# Autodesk Inventor assembly: outside-c-channel
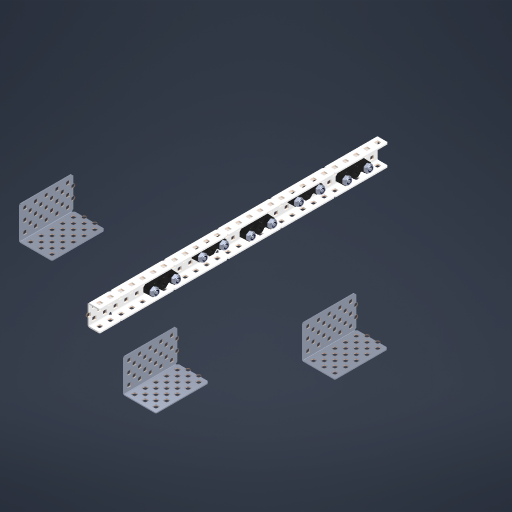
[picture p0: Inventor's stored thumbnail of the model, 512x512]
Saved by Autodesk Inventor 2023 (Build 270158000, 158)
## iProperties
Created: 2023-08-05
Part Number: outside-c-channel
Document SubType Name: Assembly
Designer: srbel
Author: srbel
## Documents named in this file (7)
- C:\CAD\OverUnderCAD\Drive\outside-c-channel.iam
- C:\CAD\OverUnderCAD\VEX-CAD-Inventor-1.4.0\Structure\C Channel\Aluminum 1x2x1\Alu C 1x2x1x27.ipt
- C:\CAD\OverUnderCAD\VEX-CAD-Inventor-1.4.0\Motion\Shaft LS\Bearing Flat.ipt
- C:\CAD\OverUnderCAD\VEX-CAD-Inventor-1.4.0\Structure\Hardware\Screw Steel - Star\SScrew Star Threaded .500.ipt
- C:\CAD\OverUnderCAD\VEX-CAD-Inventor-1.4.0\Structure\Hardware\Nut Thin Nylock.ipt
- C:\CAD\OverUnderCAD\VEX-CAD-Inventor-1.4.0\Structure\Hardware\Screw Steel - Star.ipt
- C:\CAD\OverUnderCAD\VEX-CAD-Inventor-1.4.0\Structure\Angle\Steel\3x3\Steel Angle 3x3x5.ipt
## Components (29 placed, 5 different names)
1. Alu C 1x2x1x27:2 — Insert:1, Insert:2, Insert:3, Insert:4, Insert:5, Insert:6, Insert:7, Insert:8, Insert:21, Insert:22, Insert:23, Insert:24, Insert:25, Insert:26, Insert:27, Insert:28, Insert:29, Insert:30, Insert:31, Insert:32
2. Bearing Flat:1 — Insert:1, Insert:2, Insert:41, Insert:42
3. Bearing Flat:2 — Insert:3, Insert:4, Insert:39, Insert:40
4. Bearing Flat:3 — Insert:5, Insert:6, Insert:37, Insert:38
5. Bearing Flat:4 — Insert:7, Insert:8, Insert:35, Insert:36
6. Bearing Flat:5 — Insert:21, Insert:22, Insert:33, Insert:34
7. SScrew Star Threaded .500:1 — Insert:23
8. SScrew Star Threaded .500:3 — Insert:24
9. SScrew Star Threaded .500:4 — Insert:25
10. SScrew Star Threaded .500:5 — Insert:26
11. SScrew Star Threaded .500:6 — Insert:27
12. SScrew Star Threaded .500:7 — Insert:28
13. SScrew Star Threaded .500:8 — Insert:29
14. SScrew Star Threaded .500:9 — Insert:30
15. SScrew Star Threaded .500:10 — Insert:31
16. SScrew Star Threaded .500:11 — Insert:32
17. Nut Thin Nylock:1 — Insert:33
18. Nut Thin Nylock:2 — Insert:34
19. Nut Thin Nylock:3 — Insert:35
20. Nut Thin Nylock:4 — Insert:36
21. Nut Thin Nylock:5 — Insert:37
22. Nut Thin Nylock:6 — Insert:38
23. Nut Thin Nylock:7 — Insert:39
24. Nut Thin Nylock:8 — Insert:40
25. Nut Thin Nylock:9 — Insert:41
26. Nut Thin Nylock:10 — Insert:42
27. Steel Angle 3x3x5:1
28. Steel Angle 3x3x5:2
29. Steel Angle 3x3x5:3
## Relationships (30: Insert 30)
- Insert:1: Alu C 1x2x1x27:2 ↔ Bearing Flat:1
- Insert:2: Alu C 1x2x1x27:2 ↔ Bearing Flat:1
- Insert:3: Alu C 1x2x1x27:2 ↔ Bearing Flat:2
- Insert:4: Alu C 1x2x1x27:2 ↔ Bearing Flat:2
- Insert:5: Alu C 1x2x1x27:2 ↔ Bearing Flat:3
- Insert:6: Alu C 1x2x1x27:2 ↔ Bearing Flat:3
- Insert:7: Alu C 1x2x1x27:2 ↔ Bearing Flat:4
- Insert:8: Alu C 1x2x1x27:2 ↔ Bearing Flat:4
- Insert:21: Alu C 1x2x1x27:2 ↔ Bearing Flat:5
- Insert:22: Alu C 1x2x1x27:2 ↔ Bearing Flat:5
- Insert:23: Alu C 1x2x1x27:2 ↔ SScrew Star Threaded .500:1
- Insert:24: Alu C 1x2x1x27:2 ↔ SScrew Star Threaded .500:3
- Insert:25: Alu C 1x2x1x27:2 ↔ SScrew Star Threaded .500:4
- Insert:26: Alu C 1x2x1x27:2 ↔ SScrew Star Threaded .500:5
- Insert:27: Alu C 1x2x1x27:2 ↔ SScrew Star Threaded .500:6
- Insert:28: Alu C 1x2x1x27:2 ↔ SScrew Star Threaded .500:7
- Insert:29: Alu C 1x2x1x27:2 ↔ SScrew Star Threaded .500:8
- Insert:30: Alu C 1x2x1x27:2 ↔ SScrew Star Threaded .500:9
- Insert:31: Alu C 1x2x1x27:2 ↔ SScrew Star Threaded .500:10
- Insert:32: Alu C 1x2x1x27:2 ↔ SScrew Star Threaded .500:11
- Insert:33: Bearing Flat:5 ↔ Nut Thin Nylock:1
- Insert:34: Bearing Flat:5 ↔ Nut Thin Nylock:2
- Insert:35: Bearing Flat:4 ↔ Nut Thin Nylock:3
- Insert:36: Bearing Flat:4 ↔ Nut Thin Nylock:4
- Insert:37: Bearing Flat:3 ↔ Nut Thin Nylock:5
- Insert:38: Bearing Flat:3 ↔ Nut Thin Nylock:6
- Insert:39: Bearing Flat:2 ↔ Nut Thin Nylock:7
- Insert:40: Bearing Flat:2 ↔ Nut Thin Nylock:8
- Insert:41: Bearing Flat:1 ↔ Nut Thin Nylock:9
- Insert:42: Bearing Flat:1 ↔ Nut Thin Nylock:10
